# Autodesk Inventor assembly: PerfboardBackplaneSandwichPrinthead_WithSLAPlate
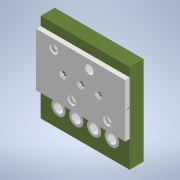
[picture p0: Inventor's stored thumbnail of the model, 180x180]
Saved by Autodesk Inventor 2021 (Build 250183000, 183)
## iProperties
Created: 2022-02-02
Part Number: PerfboardBackplaneSandwichPrinthead_WithSLAPlate
Document SubType Name: Assembly
Designer: Unit-005
Author: Unit-005
## Documents named in this file (4)
- C:\Users\Unit-005\Documents\Inventor\SiC_Monofilament_MicroheaterPrinthead\PerfboardBackplaneSandwichPrinthead_WithSLAPlate.iam
- C:\Users\Unit-005\Documents\Inventor\SiC_Monofilament_MicroheaterPrinthead\1.27mmpitchProtoboardDesign.ipt_.25inch_.25Inch.ipt
- C:\Users\Unit-005\Documents\Inventor\SiC_Monofilament_MicroheaterPrinthead\4mmSicFilamentePerfBoard.ipt
- C:\Users\Unit-005\Documents\Inventor\SiC_Monofilament_MicroheaterPrinthead\1.27mmPitchProtoboard_nozzlePlate.ipt
## Components (3 placed, 3 different names)
1. 1.27mmpitchProtoboardDesign.ipt_.25inch_.25Inch:2 — Flush:3, Tangent:1, Mate:1, Mate:2
2. 4mmSicFilamentePerfBoard:1 — Tangent:1, Mate:1, Flush:4, Flush:5
3. 1.27mmPitchProtoboard_nozzlePlate:1 — Flush:4, Mate:2, Flush:5
## Relationships (6: Flush 3, Mate 2, Tangent 1)
- Flush:3: 1.27mmpitchProtoboardDesign.ipt_.25inch_.25Inch:2
- Tangent:1: 1.27mmpitchProtoboardDesign.ipt_.25inch_.25Inch:2 ↔ 4mmSicFilamentePerfBoard:1
- Mate:1: 1.27mmpitchProtoboardDesign.ipt_.25inch_.25Inch:2 ↔ 4mmSicFilamentePerfBoard:1
- Flush:4: 4mmSicFilamentePerfBoard:1 ↔ 1.27mmPitchProtoboard_nozzlePlate:1
- Mate:2: 1.27mmpitchProtoboardDesign.ipt_.25inch_.25Inch:2 ↔ 1.27mmPitchProtoboard_nozzlePlate:1
- Flush:5: 4mmSicFilamentePerfBoard:1 ↔ 1.27mmPitchProtoboard_nozzlePlate:1
